# Autodesk Inventor assembly: shaft extender
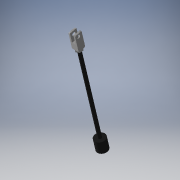
[picture p0: Inventor's stored thumbnail of the model, 180x180]
Saved by Autodesk Inventor 2017 (Build 210142000, 142)
## iProperties
Created: 2016-11-06
Part Number: shaft extender
Document SubType Name: Assembly
Designer: gus
Author: gus
## Documents named in this file (4)
- \\Mac\Home\Desktop\bunnybots 2016\15102898-16-Bunnybot-CAD\Bunnybot-To_be_renamed\15102898-16-A-0000\15102898-16-A-0900\Imported Components\AIS2015\shaft extender.iam
- \\Mac\Home\Desktop\bunnybots 2016\15102898-16-Bunnybot-CAD\Bunnybot-To_be_renamed\15102898-16-A-0000\15102898-16-A-0900\Imported Components\AIS2015\C-045-DP0_rod.ipt
- \\Mac\Home\Desktop\bunnybots 2016\15102898-16-Bunnybot-CAD\Bunnybot-To_be_renamed\15102898-16-A-0000\15102898-16-A-0900\Imported Components\AIS2015\D-14055.ipt
- \\Mac\Home\Desktop\bunnybots 2016\15102898-16-Bunnybot-CAD\Bunnybot-To_be_renamed\15102898-16-A-0000\15102898-16-A-0900\Imported Components\AIS2015\D-344.ipt
## Components (3 placed, 3 different names)
1. C-045-DP0_rod:1
2. D-14055:1
3. D-344:1
## Relationships (4: Mate 4)
- [Mate]: C-045-DP0_rod:1 ↔ D-14055:1
- [Mate]: C-045-DP0_rod:1 ↔ D-344:1
- [Mate]: C-045-DP0_rod:1 ↔ D-344:1
- [Mate]: D-14055:1 ↔ D-344:1
